# Autodesk Inventor assembly: PnP Machine
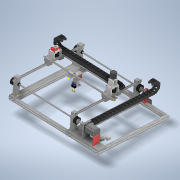
[picture p0: Inventor's stored thumbnail of the model, 180x180]
Saved by Autodesk Inventor 2020 (Build 240168000, 168)
## iProperties
Created: 2020-03-15
Part Number: PnP Machine
Document SubType Name: Assembly
Designer: DasNick
Author: DasNick
## Documents named in this file (70)
- C:\Users\DasNick\Desktop\PnP Machine\PnP Machine.iam
- C:\Users\DasNick\Desktop\PnP Machine\6061K650_HARDENED PRECISION STEEL SHAFT.ipt
- C:\Users\DasNick\Desktop\PnP Machine\1346K330_STEEL DRIVE SHAFT.ipt
- C:\Users\DasNick\Desktop\PnP Machine\47065T605_ALUMINUM T-SLOTTED FRAMING EXTRUSION.ipt
- C:\Users\DasNick\Desktop\PnP Machine\47065T415_ALUMINUM T-SLOTTED FRAMING EXTRUSION (1).ipt
- C:\Users\DasNick\Desktop\PnP Machine\BT V1.3 R2.ipt
- C:\Users\DasNick\Desktop\PnP Machine\ST8918L4508-A.ipt
- C:\Users\DasNick\Desktop\PnP Machine\ST5918L4508-A.ipt
- C:\Users\DasNick\Desktop\PnP Machine\9845T408_VIBRATE-DAMPING PRECISION FLEXIBLE SHAFT CPLG.ipt
- C:\Users\DasNick\Desktop\PnP Machine\9845T220_VIBRATE-DAMPING PRECISION FLEXIBLE SHAFT CPLG.ipt
- C:\Users\DasNick\Desktop\PnP Machine\9845T403_VIBRATE-DAMPING PRECISION FLEXIBLE SHAFT CPLG.ipt
- C:\Users\DasNick\Desktop\PnP Machine\1346K260_STEEL DRIVE SHAFT.ipt
- C:\Users\DasNick\Desktop\PnP Machine\2342K187_PERMANENTLY LUBRICATED BALL BEARING.ipt
- C:\Users\DasNick\Desktop\PnP Machine\6497K113_HIGH-STRENGTH HTD TIMING BELT PULLEY.ipt
- C:\Users\DasNick\Desktop\PnP Machine\6086K112_QUICK-DISCONNECT BUSHING.ipt
- C:\Users\DasNick\Desktop\PnP Machine\9845T204_VIBRATE-DAMPING PRECISION FLEXIBLE SHAFT CPLG.ipt
- C:\Users\DasNick\Desktop\PnP Machine\9845T201_VIBRATE-DAMPING PRECISION FLEXIBLE SHAFT CPLG.ipt
- C:\Users\DasNick\Desktop\PnP Machine\9845T150_VIBRATE-DAMPING PRECISION FLEXIBLE SHAFT CPLG.ipt
- C:\Users\DasNick\Desktop\PnP Machine\9961K190_ONE-PIECE CLAMP-ON SHAFT COLLAR.ipt
- C:\Users\DasNick\Desktop\PnP Machine\CUI_DEVICES_AMT132Q-4096-1587.ipt
- C:\Users\DasNick\Desktop\PnP Machine\CUI_DEVICES_AMT132Q-4096-1270.ipt
- C:\Users\DasNick\Desktop\PnP Machine\Head Front.ipt
- C:\Users\DasNick\Desktop\PnP Machine\Head Back.ipt
- C:\Users\DasNick\Desktop\PnP Machine\Head Rail.ipt
- C:\Users\DasNick\Desktop\PnP Machine\Corner Stands.ipt
- C:\Users\DasNick\Desktop\PnP Machine\Stand Nut.ipt
- C:\Users\DasNick\Desktop\PnP Machine\Stand Stud.ipt
- C:\Users\DasNick\Desktop\PnP Machine\Corner Stand.ipt
- C:\Users\DasNick\Desktop\PnP Machine\91251A385_BLACK-OXIDE ALLOY STEEL SOCKET HEAD CAP SCREW.ipt
- C:\Users\DasNick\Desktop\PnP Machine\9804K500_LINEAR BRNG HOUSING.ipt
- C:\Users\DasNick\Desktop\PnP Machine\6673K350_HT-SPEED LINEAR SLEEVE BRNG.ipt
- C:\Users\DasNick\Desktop\PnP Machine\6673K150_HT-SPEED LINEAR SLEEVE BRNG.ipt
- C:\Users\DasNick\Desktop\PnP Machine\YClamp.ipt
- C:\Users\DasNick\Desktop\PnP Machine\YClampTop.ipt
- C:\Users\DasNick\Desktop\PnP Machine\Transmission Clamp.ipt
- C:\Users\DasNick\Desktop\PnP Machine\Belt Clamp.ipt
- C:\Users\DasNick\Desktop\PnP Machine\5779K109_PUSH-TO-CONNECT TUBE FITTING FOR AIR.ipt
- C:\Users\DasNick\Desktop\PnP Machine\AVS-3212-24D.ipt
- C:\Users\DasNick\Desktop\PnP Machine\5779K693_PUSH-TO-CONNECT TUBE FITTING FOR AIR.ipt
- C:\Users\DasNick\Desktop\PnP Machine\47065T414_ALUMINUM T-SLOTTED FRAMING EXTRUSION.ipt
- C:\Users\DasNick\Desktop\PnP Machine\47065T415_ALUMINUM T-SLOTTED FRAMING EXTRUSION (2).ipt
- C:\Users\DasNick\Desktop\PnP Machine\4409T513_SNAP-TOGETHER CABLE AND HOSE CARRIER.ipt
- C:\Users\DasNick\Desktop\PnP Machine\Acrylic Relief Guide.ipt
- C:\Users\DasNick\Desktop\PnP Machine\Female Mounting Bracket.ipt
- C:\Users\DasNick\Desktop\PnP Machine\Male Mounting Bracket.ipt
- C:\Users\DasNick\Desktop\PnP Machine\91253A540_ALLOY STEEL FLAT-HEAD SOCKET CAP SCREW.ipt
- C:\Users\DasNick\Desktop\PnP Machine\90640A129_LOW-STRENGTH STEEL NYLON-INSERT LOCKNUT.ipt
- C:\Users\DasNick\Desktop\PnP Machine\Corner Stand Extension.ipt
- C:\Users\DasNick\Desktop\PnP Machine\Stepper Plate.ipt
- C:\Users\DasNick\Desktop\PnP Machine\Stepper Support.ipt
- C:\Users\DasNick\Desktop\PnP Machine\91251A352_BLACK-OXIDE ALLOY STEEL SOCKET HEAD SCREW.ipt
- C:\Users\DasNick\Desktop\PnP Machine\90101A225_TYPE 18-8 SS THIN NYLON-INSERT LOCKNUT (1).ipt
- C:\Users\DasNick\Desktop\PnP Machine\91251A287_BLACK-OXIDE ALLOY STEEL SOCKET HEAD SCREW.ipt
- C:\Users\DasNick\Desktop\PnP Machine\Encoder Mount 1.ipt
- C:\Users\DasNick\Desktop\PnP Machine\Head Adapter Plate.ipt
- C:\Users\DasNick\Desktop\PnP Machine\Spacer Plate.ipt
- C:\Users\DasNick\Desktop\PnP Machine\Head Spacer Plate.ipt
- C:\Users\DasNick\Desktop\PnP Machine\91290A135_BLACK-OXIDE CLASS 12.9 SOCKET HEAD CAP SCREW.ipt
- C:\Users\DasNick\Desktop\PnP Machine\Belt Clamp 2.ipt
- C:\Users\DasNick\Desktop\PnP Machine\6086K111_QUICK-DISCONNECT BUSHING.ipt
- C:\Users\DasNick\Desktop\PnP Machine\Stepper Standoff.ipt
- C:\Users\DasNick\Desktop\PnP Machine\9961K170_ONE-PIECE CLAMP-ON SHAFT COLLAR.ipt
- C:\Users\DasNick\Desktop\PnP Machine\6384K361_BALL BEARING.ipt
- C:\Users\DasNick\Desktop\PnP Machine\4768K110_SET SCREW COLLAR BALL BRNG.ipt
- C:\Users\DasNick\Desktop\PnP Machine\Stepper Mount Y.ipt
- C:\Users\DasNick\Desktop\PnP Machine\Encoder Mount Y.ipt
- C:\Users\DasNick\Desktop\PnP Machine\Steel Shaft.ipt
- C:\Users\DasNick\Desktop\PnP Machine\91251A349_BLACK-OXIDE ALLOY STEEL SOCKET HEAD SCREW.ipt
- C:\Users\DasNick\Desktop\PnP Machine\Printed Encoder Mount.ipt
- C:\Users\DasNick\Desktop\PnP Machine\Stepper Spacer Y.ipt
## Components (226 placed, 69 different names)
1. 6061K650_HARDENED PRECISION STEEL SHAFT:1
2. 6061K650_HARDENED PRECISION STEEL SHAFT:2
3. 47065T605_ALUMINUM T-SLOTTED FRAMING EXTRUSION:1
4. 47065T605_ALUMINUM T-SLOTTED FRAMING EXTRUSION:2
5. 47065T415_ALUMINUM T-SLOTTED FRAMING EXTRUSION (1):1
6. 47065T415_ALUMINUM T-SLOTTED FRAMING EXTRUSION (1):2
7. BT V1.3 R2:1
8. ST8918L4508-A:1
9. ST5918L4508-A:1 — Mate:10, Mate:11, Mate:12, Mate:13, Mate:14
10. 9845T408_VIBRATE-DAMPING PRECISION FLEXIBLE SHAFT CPLG:2
11. 9845T220_VIBRATE-DAMPING PRECISION FLEXIBLE SHAFT CPLG:1
12. 9845T403_VIBRATE-DAMPING PRECISION FLEXIBLE SHAFT CPLG:1
13. 1346K260_STEEL DRIVE SHAFT:1
14. 2342K187_PERMANENTLY LUBRICATED BALL BEARING:1
15. 6497K113_HIGH-STRENGTH HTD TIMING BELT PULLEY:1
16. 6086K112_QUICK-DISCONNECT BUSHING:1
17. 6497K113_HIGH-STRENGTH HTD TIMING BELT PULLEY:5
18. 6086K112_QUICK-DISCONNECT BUSHING:5
19. 9845T204_VIBRATE-DAMPING PRECISION FLEXIBLE SHAFT CPLG:1
20. 9845T201_VIBRATE-DAMPING PRECISION FLEXIBLE SHAFT CPLG:1
21. 9845T150_VIBRATE-DAMPING PRECISION FLEXIBLE SHAFT CPLG:1
22. 1346K260_STEEL DRIVE SHAFT:2
23. 6497K113_HIGH-STRENGTH HTD TIMING BELT PULLEY:7
24. 6086K112_QUICK-DISCONNECT BUSHING:7
25. 6497K113_HIGH-STRENGTH HTD TIMING BELT PULLEY:8
26. 6086K112_QUICK-DISCONNECT BUSHING:8
27. 9961K190_ONE-PIECE CLAMP-ON SHAFT COLLAR:1
28. 9961K190_ONE-PIECE CLAMP-ON SHAFT COLLAR:2
29. 9961K190_ONE-PIECE CLAMP-ON SHAFT COLLAR:3
30. 9961K190_ONE-PIECE CLAMP-ON SHAFT COLLAR:4
31. CUI_DEVICES_AMT132Q-4096-1587:1
32. CUI_DEVICES_AMT132Q-4096-1270:1
33. Head Front:1
34. Head Back:1
35. Head Rail:1
36. Head Rail:2
37. Corner Stands:1
38. Stand Nut:1
39. Stand Stud:1
40. Stand Nut:2
41. Stand Nut:3
42. Stand Nut:4
43. Stand Stud:2
44. Stand Stud:3
45. Stand Stud:4
46. Corner Stand:1
47. 91251A385_BLACK-OXIDE ALLOY STEEL SOCKET HEAD CAP SCREW:1
48. 91251A385_BLACK-OXIDE ALLOY STEEL SOCKET HEAD CAP SCREW:2
49. 91251A385_BLACK-OXIDE ALLOY STEEL SOCKET HEAD CAP SCREW:3
50. 91251A385_BLACK-OXIDE ALLOY STEEL SOCKET HEAD CAP SCREW:4
51. 91251A385_BLACK-OXIDE ALLOY STEEL SOCKET HEAD CAP SCREW:5
52. 91251A385_BLACK-OXIDE ALLOY STEEL SOCKET HEAD CAP SCREW:6
53. 2342K187_PERMANENTLY LUBRICATED BALL BEARING:3
54. Stand Nut:5
55. Stand Nut:6
56. Stand Nut:7
57. Stand Nut:8
58. Corner Stand:2
59. 91251A385_BLACK-OXIDE ALLOY STEEL SOCKET HEAD CAP SCREW:7
60. 91251A385_BLACK-OXIDE ALLOY STEEL SOCKET HEAD CAP SCREW:8
61. 91251A385_BLACK-OXIDE ALLOY STEEL SOCKET HEAD CAP SCREW:9
62. 91251A385_BLACK-OXIDE ALLOY STEEL SOCKET HEAD CAP SCREW:10
63. 91251A385_BLACK-OXIDE ALLOY STEEL SOCKET HEAD CAP SCREW:11
64. 91251A385_BLACK-OXIDE ALLOY STEEL SOCKET HEAD CAP SCREW:12
65. 2342K187_PERMANENTLY LUBRICATED BALL BEARING:4
66. Corner Stands:3
67. Stand Nut:9
68. Stand Nut:10
69. Stand Nut:11
70. Stand Nut:12
71. Corner Stand:3
72. 91251A385_BLACK-OXIDE ALLOY STEEL SOCKET HEAD CAP SCREW:13
73. 91251A385_BLACK-OXIDE ALLOY STEEL SOCKET HEAD CAP SCREW:14
74. 91251A385_BLACK-OXIDE ALLOY STEEL SOCKET HEAD CAP SCREW:15
75. 91251A385_BLACK-OXIDE ALLOY STEEL SOCKET HEAD CAP SCREW:16
76. 91251A385_BLACK-OXIDE ALLOY STEEL SOCKET HEAD CAP SCREW:17
77. 91251A385_BLACK-OXIDE ALLOY STEEL SOCKET HEAD CAP SCREW:18
78. 2342K187_PERMANENTLY LUBRICATED BALL BEARING:5
79. Corner Stands:4
80. Stand Nut:13
81. Stand Nut:14
82. Stand Nut:15
83. Stand Nut:16
84. Corner Stand:4
85. 91251A385_BLACK-OXIDE ALLOY STEEL SOCKET HEAD CAP SCREW:19
86. 91251A385_BLACK-OXIDE ALLOY STEEL SOCKET HEAD CAP SCREW:20
87. 91251A385_BLACK-OXIDE ALLOY STEEL SOCKET HEAD CAP SCREW:21
88. 91251A385_BLACK-OXIDE ALLOY STEEL SOCKET HEAD CAP SCREW:22
89. 91251A385_BLACK-OXIDE ALLOY STEEL SOCKET HEAD CAP SCREW:23
90. 91251A385_BLACK-OXIDE ALLOY STEEL SOCKET HEAD CAP SCREW:24
91. 1346K330_STEEL DRIVE SHAFT:2
92. 9804K500_LINEAR BRNG HOUSING:3
93. 6673K350_HT-SPEED LINEAR SLEEVE BRNG:2
94. 9804K500_LINEAR BRNG HOUSING:4
95. 6673K350_HT-SPEED LINEAR SLEEVE BRNG:3
96. 9804K500_LINEAR BRNG HOUSING:7
97. 6673K350_HT-SPEED LINEAR SLEEVE BRNG:4
98. 9804K500_LINEAR BRNG HOUSING:8
99. 6673K350_HT-SPEED LINEAR SLEEVE BRNG:5
100. YClamp:1 — Mate:1, Mate:2, Mate:3, Mate:8, Mate:9
101. YClampTop:1
102. YClampTop:2
103. Transmission Clamp:1
104. Belt Clamp:1
105. YClamp:2 — Mate:4, Mate:5, Mate:6, Mate:7
106. YClampTop:3
107. YClampTop:4
108. Transmission Clamp:2
109. Belt Clamp:2
110. 1346K330_STEEL DRIVE SHAFT:3
111. 5779K109_PUSH-TO-CONNECT TUBE FITTING FOR AIR:1
112. 5779K109_PUSH-TO-CONNECT TUBE FITTING FOR AIR:2
113. 5779K109_PUSH-TO-CONNECT TUBE FITTING FOR AIR:3
114. 5779K109_PUSH-TO-CONNECT TUBE FITTING FOR AIR:4
115. 5779K109_PUSH-TO-CONNECT TUBE FITTING FOR AIR:5
116. 5779K109_PUSH-TO-CONNECT TUBE FITTING FOR AIR:6
117. AVS-3212-24D:1
118. AVS-3212-24D:2
119. 5779K693_PUSH-TO-CONNECT TUBE FITTING FOR AIR:1
120. 47065T414_ALUMINUM T-SLOTTED FRAMING EXTRUSION:1
121. 47065T414_ALUMINUM T-SLOTTED FRAMING EXTRUSION:2
122. 47065T415_ALUMINUM T-SLOTTED FRAMING EXTRUSION (2):1
123. 4409T513_SNAP-TOGETHER CABLE AND HOSE CARRIER:1
124. Acrylic Relief Guide:1
125. Female Mounting Bracket:1
126. Male Mounting Bracket:1
127. 4409T513_SNAP-TOGETHER CABLE AND HOSE CARRIER:2
128. Female Mounting Bracket:2
129. Male Mounting Bracket:2
130. 91253A540_ALLOY STEEL FLAT-HEAD SOCKET CAP SCREW:1
131. 91253A540_ALLOY STEEL FLAT-HEAD SOCKET CAP SCREW:2
132. 90640A129_LOW-STRENGTH STEEL NYLON-INSERT LOCKNUT:1
133. 90640A129_LOW-STRENGTH STEEL NYLON-INSERT LOCKNUT:2
134. Corner Stand Extension:1
135. Stepper Plate:1
136. Stepper Support:1
137. 91251A352_BLACK-OXIDE ALLOY STEEL SOCKET HEAD SCREW:1
138. 91251A352_BLACK-OXIDE ALLOY STEEL SOCKET HEAD SCREW:2
139. 90101A225_TYPE 18-8 SS THIN NYLON-INSERT LOCKNUT (1):1
140. 90101A225_TYPE 18-8 SS THIN NYLON-INSERT LOCKNUT (1):2
141. 90101A225_TYPE 18-8 SS THIN NYLON-INSERT LOCKNUT (1):3
142. 90101A225_TYPE 18-8 SS THIN NYLON-INSERT LOCKNUT (1):4
143. 91251A352_BLACK-OXIDE ALLOY STEEL SOCKET HEAD SCREW:3
144. 91251A352_BLACK-OXIDE ALLOY STEEL SOCKET HEAD SCREW:4
145. 91251A352_BLACK-OXIDE ALLOY STEEL SOCKET HEAD SCREW:5
146. 91251A352_BLACK-OXIDE ALLOY STEEL SOCKET HEAD SCREW:6
147. 91251A352_BLACK-OXIDE ALLOY STEEL SOCKET HEAD SCREW:7
148. 91251A352_BLACK-OXIDE ALLOY STEEL SOCKET HEAD SCREW:8
149. 91251A352_BLACK-OXIDE ALLOY STEEL SOCKET HEAD SCREW:9
150. 91251A352_BLACK-OXIDE ALLOY STEEL SOCKET HEAD SCREW:10
151. 90101A225_TYPE 18-8 SS THIN NYLON-INSERT LOCKNUT (1):5
152. 90101A225_TYPE 18-8 SS THIN NYLON-INSERT LOCKNUT (1):6
153. 90101A225_TYPE 18-8 SS THIN NYLON-INSERT LOCKNUT (1):7
154. 90101A225_TYPE 18-8 SS THIN NYLON-INSERT LOCKNUT (1):8
155. 91251A352_BLACK-OXIDE ALLOY STEEL SOCKET HEAD SCREW:11
156. 91251A352_BLACK-OXIDE ALLOY STEEL SOCKET HEAD SCREW:12
157. 91251A352_BLACK-OXIDE ALLOY STEEL SOCKET HEAD SCREW:13
158. 91251A352_BLACK-OXIDE ALLOY STEEL SOCKET HEAD SCREW:14
159. 91251A352_BLACK-OXIDE ALLOY STEEL SOCKET HEAD SCREW:15
160. 91251A352_BLACK-OXIDE ALLOY STEEL SOCKET HEAD SCREW:16
161. 91251A287_BLACK-OXIDE ALLOY STEEL SOCKET HEAD SCREW:1
162. 91251A287_BLACK-OXIDE ALLOY STEEL SOCKET HEAD SCREW:2
163. 91251A287_BLACK-OXIDE ALLOY STEEL SOCKET HEAD SCREW:3
164. 91251A287_BLACK-OXIDE ALLOY STEEL SOCKET HEAD SCREW:4
165. 91251A287_BLACK-OXIDE ALLOY STEEL SOCKET HEAD SCREW:5
166. 91251A287_BLACK-OXIDE ALLOY STEEL SOCKET HEAD SCREW:6
167. Encoder Mount 1:1
168. 9804K500_LINEAR BRNG HOUSING:9
169. 6673K150_HT-SPEED LINEAR SLEEVE BRNG:2
170. 9804K500_LINEAR BRNG HOUSING:11
171. 6673K150_HT-SPEED LINEAR SLEEVE BRNG:4
172. Head Adapter Plate:1
173. Spacer Plate:1
174. Head Spacer Plate:1
175. 90101A225_TYPE 18-8 SS THIN NYLON-INSERT LOCKNUT (1):9
176. 90101A225_TYPE 18-8 SS THIN NYLON-INSERT LOCKNUT (1):10
177. 90101A225_TYPE 18-8 SS THIN NYLON-INSERT LOCKNUT (1):11
178. 90101A225_TYPE 18-8 SS THIN NYLON-INSERT LOCKNUT (1):12
179. Belt Clamp 2:1
180. 91290A135_BLACK-OXIDE CLASS 12.9 SOCKET HEAD CAP SCREW:2
181. 91290A135_BLACK-OXIDE CLASS 12.9 SOCKET HEAD CAP SCREW:3
182. 91290A135_BLACK-OXIDE CLASS 12.9 SOCKET HEAD CAP SCREW:4
183. 91290A135_BLACK-OXIDE CLASS 12.9 SOCKET HEAD CAP SCREW:5
184. 6497K113_HIGH-STRENGTH HTD TIMING BELT PULLEY:9
185. 6497K113_HIGH-STRENGTH HTD TIMING BELT PULLEY:10
186. 6086K111_QUICK-DISCONNECT BUSHING:1
187. 6086K111_QUICK-DISCONNECT BUSHING:2
188. Stepper Standoff:1
189. 9961K170_ONE-PIECE CLAMP-ON SHAFT COLLAR:1
190. 6384K361_BALL BEARING:1
191. 6384K361_BALL BEARING:3
192. 6384K361_BALL BEARING:4
193. Stepper Standoff:2
194. Stepper Standoff:3
195. Stepper Standoff:4
196. 4768K110_SET SCREW COLLAR BALL BRNG:1
197. Stepper Mount Y:1 — Flush:9
198. Encoder Mount Y:1 — Flush:8
199. Steel Shaft:1
200. Steel Shaft:2
201. 91251A349_BLACK-OXIDE ALLOY STEEL SOCKET HEAD SCREW:1
202. 91251A349_BLACK-OXIDE ALLOY STEEL SOCKET HEAD SCREW:2
203. 91251A349_BLACK-OXIDE ALLOY STEEL SOCKET HEAD SCREW:3
204. 91251A349_BLACK-OXIDE ALLOY STEEL SOCKET HEAD SCREW:4
205. 91251A349_BLACK-OXIDE ALLOY STEEL SOCKET HEAD SCREW:5
206. 91251A349_BLACK-OXIDE ALLOY STEEL SOCKET HEAD SCREW:6
207. 91251A349_BLACK-OXIDE ALLOY STEEL SOCKET HEAD SCREW:7
208. 91251A349_BLACK-OXIDE ALLOY STEEL SOCKET HEAD SCREW:8
209. 91251A349_BLACK-OXIDE ALLOY STEEL SOCKET HEAD SCREW:9 — Mate:4, Flush:7
210. 91251A349_BLACK-OXIDE ALLOY STEEL SOCKET HEAD SCREW:10 — Mate:3, Flush:2, Flush:3
211. 91251A349_BLACK-OXIDE ALLOY STEEL SOCKET HEAD SCREW:11 — Mate:2, Flush:3, Flush:4
212. 91251A349_BLACK-OXIDE ALLOY STEEL SOCKET HEAD SCREW:12 — Mate:1, Flush:1
213. 91251A349_BLACK-OXIDE ALLOY STEEL SOCKET HEAD SCREW:13 — Mate:5, Flush:4, Flush:5
214. 91251A349_BLACK-OXIDE ALLOY STEEL SOCKET HEAD SCREW:14 — Mate:6, Flush:6, Flush:7
215. 91251A349_BLACK-OXIDE ALLOY STEEL SOCKET HEAD SCREW:15 — Mate:7, Flush:5, Flush:6
216. 91251A349_BLACK-OXIDE ALLOY STEEL SOCKET HEAD SCREW:16 — Mate:8, Mate:9, Flush:1, Flush:2
217. Printed Encoder Mount:1 — Flush:8, Mate:15, Mate:16, Mate:17, Mate:18, Mate:19
218. Stepper Spacer Y:1 — Flush:9
219. 91251A349_BLACK-OXIDE ALLOY STEEL SOCKET HEAD SCREW:17 — Flush:11, Flush:12, Mate:12
220. 91251A349_BLACK-OXIDE ALLOY STEEL SOCKET HEAD SCREW:18 — Flush:12, Mate:13
221. 91251A349_BLACK-OXIDE ALLOY STEEL SOCKET HEAD SCREW:19 — Flush:10, Flush:11, Mate:14
222. 91251A349_BLACK-OXIDE ALLOY STEEL SOCKET HEAD SCREW:20 — Flush:10, Mate:10, Mate:11
223. 91251A349_BLACK-OXIDE ALLOY STEEL SOCKET HEAD SCREW:21 — Mate:15, Mate:16, Flush:15
224. 91251A349_BLACK-OXIDE ALLOY STEEL SOCKET HEAD SCREW:22 — Flush:14, Mate:19
225. 91251A349_BLACK-OXIDE ALLOY STEEL SOCKET HEAD SCREW:23 — Flush:13, Flush:14, Mate:18
226. 91251A349_BLACK-OXIDE ALLOY STEEL SOCKET HEAD SCREW:24 — Flush:13, Flush:15, Mate:17
## Relationships (34: Mate 19, Flush 15)
- Mate:1: YClamp:1 ↔ 91251A349_BLACK-OXIDE ALLOY STEEL SOCKET HEAD SCREW:12
- Mate:2: YClamp:1 ↔ 91251A349_BLACK-OXIDE ALLOY STEEL SOCKET HEAD SCREW:11
- Mate:3: YClamp:1 ↔ 91251A349_BLACK-OXIDE ALLOY STEEL SOCKET HEAD SCREW:10
- Mate:4: YClamp:2 ↔ 91251A349_BLACK-OXIDE ALLOY STEEL SOCKET HEAD SCREW:9
- Mate:5: YClamp:2 ↔ 91251A349_BLACK-OXIDE ALLOY STEEL SOCKET HEAD SCREW:13
- Mate:6: YClamp:2 ↔ 91251A349_BLACK-OXIDE ALLOY STEEL SOCKET HEAD SCREW:14
- Mate:7: YClamp:2 ↔ 91251A349_BLACK-OXIDE ALLOY STEEL SOCKET HEAD SCREW:15
- Mate:8: YClamp:1 ↔ 91251A349_BLACK-OXIDE ALLOY STEEL SOCKET HEAD SCREW:16
- Mate:9: YClamp:1 ↔ 91251A349_BLACK-OXIDE ALLOY STEEL SOCKET HEAD SCREW:16
- Flush:1: 91251A349_BLACK-OXIDE ALLOY STEEL SOCKET HEAD SCREW:12 ↔ 91251A349_BLACK-OXIDE ALLOY STEEL SOCKET HEAD SCREW:16
- Flush:2: 91251A349_BLACK-OXIDE ALLOY STEEL SOCKET HEAD SCREW:10 ↔ 91251A349_BLACK-OXIDE ALLOY STEEL SOCKET HEAD SCREW:16
- Flush:3: 91251A349_BLACK-OXIDE ALLOY STEEL SOCKET HEAD SCREW:10 ↔ 91251A349_BLACK-OXIDE ALLOY STEEL SOCKET HEAD SCREW:11
- Flush:4: 91251A349_BLACK-OXIDE ALLOY STEEL SOCKET HEAD SCREW:11 ↔ 91251A349_BLACK-OXIDE ALLOY STEEL SOCKET HEAD SCREW:13
- Flush:5: 91251A349_BLACK-OXIDE ALLOY STEEL SOCKET HEAD SCREW:13 ↔ 91251A349_BLACK-OXIDE ALLOY STEEL SOCKET HEAD SCREW:15
- Flush:6: 91251A349_BLACK-OXIDE ALLOY STEEL SOCKET HEAD SCREW:14 ↔ 91251A349_BLACK-OXIDE ALLOY STEEL SOCKET HEAD SCREW:15
- Flush:7: 91251A349_BLACK-OXIDE ALLOY STEEL SOCKET HEAD SCREW:9 ↔ 91251A349_BLACK-OXIDE ALLOY STEEL SOCKET HEAD SCREW:14
- Flush:8: Encoder Mount Y:1 ↔ Printed Encoder Mount:1
- Flush:9: Stepper Mount Y:1 ↔ Stepper Spacer Y:1
- Flush:10: 91251A349_BLACK-OXIDE ALLOY STEEL SOCKET HEAD SCREW:19 ↔ 91251A349_BLACK-OXIDE ALLOY STEEL SOCKET HEAD SCREW:20
- Flush:11: 91251A349_BLACK-OXIDE ALLOY STEEL SOCKET HEAD SCREW:17 ↔ 91251A349_BLACK-OXIDE ALLOY STEEL SOCKET HEAD SCREW:19
- Flush:12: 91251A349_BLACK-OXIDE ALLOY STEEL SOCKET HEAD SCREW:17 ↔ 91251A349_BLACK-OXIDE ALLOY STEEL SOCKET HEAD SCREW:18
- Mate:10: ST5918L4508-A:1 ↔ 91251A349_BLACK-OXIDE ALLOY STEEL SOCKET HEAD SCREW:20
- Mate:11: ST5918L4508-A:1 ↔ 91251A349_BLACK-OXIDE ALLOY STEEL SOCKET HEAD SCREW:20
- Mate:12: ST5918L4508-A:1 ↔ 91251A349_BLACK-OXIDE ALLOY STEEL SOCKET HEAD SCREW:17
- Mate:13: ST5918L4508-A:1 ↔ 91251A349_BLACK-OXIDE ALLOY STEEL SOCKET HEAD SCREW:18
- Mate:14: ST5918L4508-A:1 ↔ 91251A349_BLACK-OXIDE ALLOY STEEL SOCKET HEAD SCREW:19
- Mate:15: Printed Encoder Mount:1 ↔ 91251A349_BLACK-OXIDE ALLOY STEEL SOCKET HEAD SCREW:21
- Mate:16: Printed Encoder Mount:1 ↔ 91251A349_BLACK-OXIDE ALLOY STEEL SOCKET HEAD SCREW:21
- Flush:13: 91251A349_BLACK-OXIDE ALLOY STEEL SOCKET HEAD SCREW:23 ↔ 91251A349_BLACK-OXIDE ALLOY STEEL SOCKET HEAD SCREW:24
- Flush:14: 91251A349_BLACK-OXIDE ALLOY STEEL SOCKET HEAD SCREW:22 ↔ 91251A349_BLACK-OXIDE ALLOY STEEL SOCKET HEAD SCREW:23
- Flush:15: 91251A349_BLACK-OXIDE ALLOY STEEL SOCKET HEAD SCREW:21 ↔ 91251A349_BLACK-OXIDE ALLOY STEEL SOCKET HEAD SCREW:24
- Mate:17: Printed Encoder Mount:1 ↔ 91251A349_BLACK-OXIDE ALLOY STEEL SOCKET HEAD SCREW:24
- Mate:18: Printed Encoder Mount:1 ↔ 91251A349_BLACK-OXIDE ALLOY STEEL SOCKET HEAD SCREW:23
- Mate:19: Printed Encoder Mount:1 ↔ 91251A349_BLACK-OXIDE ALLOY STEEL SOCKET HEAD SCREW:22
